# Autodesk Inventor assembly: Spark Max With Mount
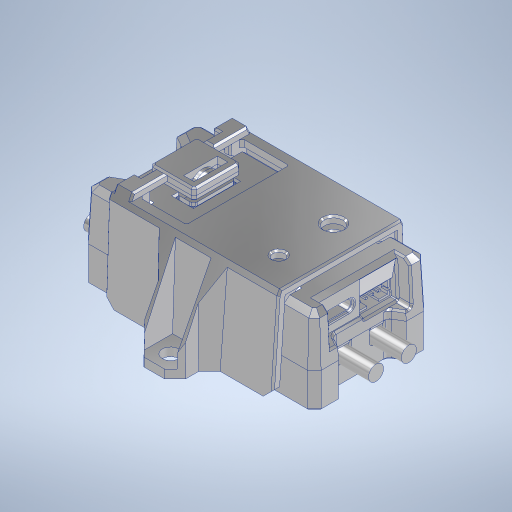
[picture p0: Inventor's stored thumbnail of the model, 512x512]
Saved by Autodesk Inventor 2023 (Build 270158000, 158)
## iProperties
Created: 2024-02-02
Part Number: Spark Max With Mount
Document SubType Name: Assembly
Designer: slick
Author: slick
## Documents named in this file (3)
- C:\Users\slick\OneDrive\Desktop\Crescendo_2024-CAD\2024 Robot\COMMON PARTS\MOTOR CONTROLERS\Spark Max With Mount.iam
- C:\Users\slick\OneDrive\Desktop\Crescendo_2024-CAD\2024 Robot\COMMON PARTS\MOTOR CONTROLERS\Spark MaxREV-11-2158.ipt
- C:\Users\slick\OneDrive\Desktop\Crescendo_2024-CAD\2024 Robot\COMMON PARTS\MOTOR CONTROLERS\Spark Max Mount PlateREV-21-2151.ipt
## Components (2 placed, 2 different names)
1. Spark MaxREV-11-2158:1 — Flush:1, Mate:1, Mate:2
2. Spark Max Mount PlateREV-21-2151:1 — Flush:1, Mate:1, Mate:2
## Relationships (3: Mate 2, Flush 1)
- Flush:1: Spark MaxREV-11-2158:1 ↔ Spark Max Mount PlateREV-21-2151:1
- Mate:1: Spark MaxREV-11-2158:1 ↔ Spark Max Mount PlateREV-21-2151:1
- Mate:2: Spark MaxREV-11-2158:1 ↔ Spark Max Mount PlateREV-21-2151:1
